# Autodesk Inventor assembly: PZT Assembly
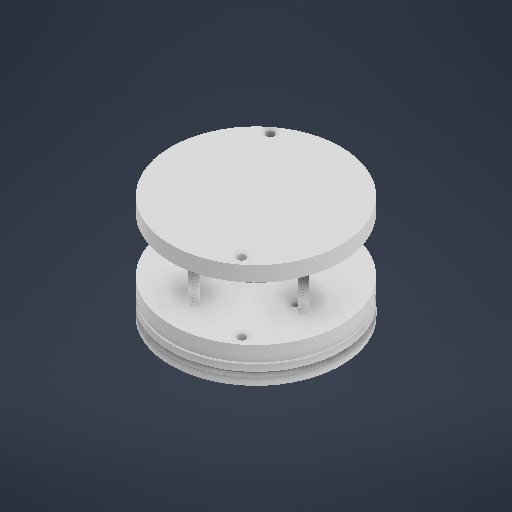
[picture p0: Inventor's stored thumbnail of the model, 512x512]
Saved by Autodesk Inventor 2025 (Build 290162000, 162)
## iProperties
Created: 2024-07-01
Part Number: PZT Assembly
Document SubType Name: Assembly
Designer: mayhe
Author: mayhe
## Documents named in this file (9)
- C:\Users\mayhe\OneDrive\Documents\GitHub\In-situ-monitoring-of-powder-bed-fusion-additive-manufacturing\system_development\Orichalcum\v0.2\Hardware_design\pzt-parts\PZT Assembly.iam
- C:\Users\mayhe\OneDrive\Documents\GitHub\In-situ-monitoring-of-powder-bed-fusion-additive-manufacturing\system_development\Orichalcum\v0.2\Hardware_design\pzt-parts\shaker.ipt
- C:\Users\mayhe\OneDrive\Documents\GitHub\In-situ-monitoring-of-powder-bed-fusion-additive-manufacturing\system_development\Orichalcum\v0.2\Hardware_design\pzt-parts\Modified Substrate Plate Bottom.ipt
- C:\Users\mayhe\OneDrive\Documents\GitHub\In-situ-monitoring-of-powder-bed-fusion-additive-manufacturing\system_development\Orichalcum\v0.2\Hardware_design\pzt-parts\shaker cut.ipt
- C:\Users\mayhe\OneDrive\Documents\GitHub\In-situ-monitoring-of-powder-bed-fusion-additive-manufacturing\system_development\Orichalcum\v0.2\Hardware_design\pzt-parts\Build Plateform.ipt
- C:\Users\mayhe\OneDrive\Documents\GitHub\In-situ-monitoring-of-powder-bed-fusion-additive-manufacturing\system_development\Orichalcum\v0.2\Hardware_design\pzt-parts\Clamp Ring.ipt
- C:\Users\mayhe\OneDrive\Documents\GitHub\In-situ-monitoring-of-powder-bed-fusion-additive-manufacturing\system_development\Orichalcum\v0.2\Hardware_design\pzt-parts\substrate plate 12mm hole.ipt
- C:\Users\mayhe\OneDrive\Documents\GitHub\In-situ-monitoring-of-powder-bed-fusion-additive-manufacturing\system_development\Orichalcum\v0.2\Hardware_design\pzt-parts\91292A229_18-8 Stainless Steel Socket Head Sc.ipt
- C:\Users\mayhe\OneDrive\Documents\GitHub\In-situ-monitoring-of-powder-bed-fusion-additive-manufacturing\system_development\Orichalcum\v0.2\Hardware_design\pzt-parts\1078N152_Class 10.9 High-Strength Steel Threa.ipt
## Components (12 placed, 8 different names)
1. shaker:1 — Rotational:2
2. Modified Substrate Plate Bottom:1 — Rotational:2
3. shaker cut:1 — Rotational:4, Rotational:5
4. Build Plateform:1 — Mate:1, Rotational:3, Rotational:6
5. Clamp Ring:1 — Mate:1, Rotational:3
6. substrate plate 12mm hole:1 — Rotational:4, Rotational:7, Mate:2
7. 91292A229_18-8 Stainless Steel Socket Head Sc:1 — Rotational:5
8. Modified Substrate Plate Bottom:3 — Rotational:6, Rigid:1, Rigid:2, Rigid:3, Rigid:4
9. 1078N152_Class 10.9 High-Strength Steel Threa:1 — Rigid:1, Rotational:7
10. 1078N152_Class 10.9 High-Strength Steel Threa:2 — Rigid:2
11. 1078N152_Class 10.9 High-Strength Steel Threa:3 — Rigid:3
12. 1078N152_Class 10.9 High-Strength Steel Threa:4 — Rigid:4, Mate:2
## Relationships (12: RevoluteJoint 6, WeldJoint 4, Mate 2)
- Rotational:2 [RevoluteJoint]: shaker:1 ↔ Modified Substrate Plate Bottom:1
- Mate:1: Build Plateform:1 ↔ Clamp Ring:1
- Rotational:3 [RevoluteJoint]: Build Plateform:1 ↔ Clamp Ring:1
- Rotational:4 [RevoluteJoint]: shaker cut:1 ↔ substrate plate 12mm hole:1
- Rotational:5 [RevoluteJoint]: shaker cut:1 ↔ 91292A229_18-8 Stainless Steel Socket Head Sc:1
- Rotational:6 [RevoluteJoint]: Build Plateform:1 ↔ Modified Substrate Plate Bottom:3
- Rigid:1 [WeldJoint]: Modified Substrate Plate Bottom:3 ↔ 1078N152_Class 10.9 High-Strength Steel Threa:1
- Rigid:2 [WeldJoint]: Modified Substrate Plate Bottom:3 ↔ 1078N152_Class 10.9 High-Strength Steel Threa:2
- Rigid:3 [WeldJoint]: Modified Substrate Plate Bottom:3 ↔ 1078N152_Class 10.9 High-Strength Steel Threa:3
- Rigid:4 [WeldJoint]: Modified Substrate Plate Bottom:3 ↔ 1078N152_Class 10.9 High-Strength Steel Threa:4
- Rotational:7 [RevoluteJoint]: substrate plate 12mm hole:1 ↔ 1078N152_Class 10.9 High-Strength Steel Threa:1
- Mate:2: substrate plate 12mm hole:1 ↔ 1078N152_Class 10.9 High-Strength Steel Threa:4
